# Autodesk Inventor assembly: Assembly1 of ROV O-ring fitting
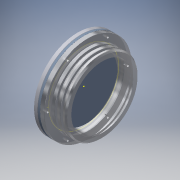
[picture p0: Inventor's stored thumbnail of the model, 180x180]
Saved by Autodesk Inventor 2016 (Build 200138000, 138)
## iProperties
Created: 2017-09-27
Part Number: Assembly1 of ROV O-ring fitting
Document SubType Name: Assembly
Designer: Student
Author: Student
## Documents named in this file (4)
- C:\Users\Student\Downloads\Assembly1 of ROV O-ring fitting.iam
- C:\Users\Student\Downloads\Oring Fitting Dome V1 end part.ipt
- C:\Users\Student\Downloads\Acrylic lense.ipt
- C:\Users\Student\Downloads\Oring Fitting Dome V2 -part.ipt
## Components (3 placed, 3 different names)
1. Oring Fitting Dome V1 end part:1 — Rigid:1
2. Acrylic lense:1 — Rigid:1, Rotational:1
3. Oring Fitting Dome V2 -part:1 — Rotational:1
## Relationships (2: WeldJoint 1, RevoluteJoint 1)
- Rigid:1 [WeldJoint]: Oring Fitting Dome V1 end part:1 ↔ Acrylic lense:1
- Rotational:1 [RevoluteJoint]: Acrylic lense:1 ↔ Oring Fitting Dome V2 -part:1
